# Autodesk Inventor assembly: motor_set
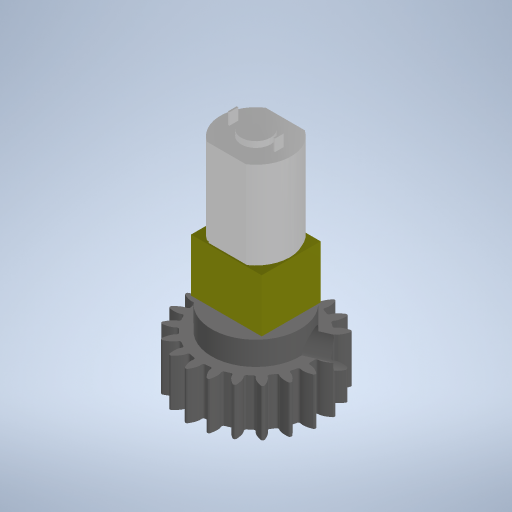
[picture p0: Inventor's stored thumbnail of the model, 512x512]
Saved by Autodesk Inventor 2024.1 (Build 281209000, 209)
## iProperties
Created: 2025-01-18
Part Number: motor_set
Document SubType Name: Assembly
Designer: hibik
Author: hibik
## Documents named in this file (5)
- C:\Users\hibik\Documents\Robomech\RESCUE\ORCA\hard\fork\fork\motor_set.iam
- C:\Users\hibik\Documents\Robomech\RESCUE\ORCA\hard\std_parts\motor_6V_60RPM.ipt
- C:\Users\hibik\Documents\Robomech\RESCUE\ORCA\hard\fork\fork\screw_bearing_setter.ipt
- C:\Users\hibik\Documents\Robomech\RESCUE\ORCA\hard\std_parts\bearing_6_10_3.ipt
- C:\Users\hibik\Documents\Robomech\RESCUE\ORCA\hard\fork\fork\screw_gear_under.ipt
## Components (4 placed, 4 different names)
1. motor_6V_60RPM:1 — 挿入:3
2. screw_bearing_setter:1 — 挿入:2, 挿入:3
3. screw_gear_under:1 — 挿入:1
4. bearing_6_10_3:1 — 挿入:1, 挿入:2
## Relationships (3: Insert 3)
- 挿入:1 [Insert]: screw_gear_under:1 ↔ bearing_6_10_3:1
- 挿入:2 [Insert]: screw_bearing_setter:1 ↔ bearing_6_10_3:1
- 挿入:3 [Insert]: motor_6V_60RPM:1 ↔ screw_bearing_setter:1
